# Autodesk Inventor assembly: pinionForRyobiPart
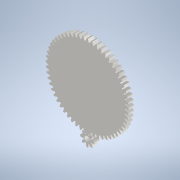
[picture p0: Inventor's stored thumbnail of the model, 180x180]
Saved by Autodesk Inventor 2022.2 (Build 262287010, 287A)
## iProperties
Created: 2022-08-10
Part Number: pinionForRyobiPart
Document SubType Name: Assembly
Designer: robst
Author: robst
## Documents named in this file (3)
- C:\git\CAD-Development\robSteele\pinionForRyobiPart.iam
- C:\git\CAD-Development\robSteele\pinionForRyobiPart.ipt
- C:\git\CAD-Development\robSteele\pinionForRyobiPart\Design Accelerator\Spur Gears1.iam
## Components (2 placed, 2 different names)
1. pinionForRyobiPart:1 — Mate:1
2. Spur Gears:1 [sub-assembly] — Mate:1
## Relationships (1: Mate 1)
- Mate:1: pinionForRyobiPart:1 ↔ Spur Gears:1
